# Autodesk Inventor assembly: Roller Assembly 1764
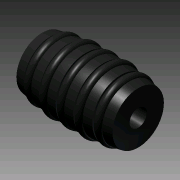
[picture p0: Inventor's stored thumbnail of the model, 180x180]
Saved by Autodesk Inventor 2011 (Build 150239000, 239)
## iProperties
Created: 2007-11-29
Part Number: Roller Assembly 1764
Document SubType Name: Assembly
Designer: lwoods
Author: lwoods
## Documents named in this file (4)
- R:\CAD Archives\Wheels\Omniwheel 1764\Roller Assembly 1764.iam
- R:\CAD Archives\Wheels\Omniwheel 1764\RollerRidges 1764.ipt
- R:\CAD Archives\Wheels\Omniwheel 1764\O Ring 1 R.609 1764.ipt
- R:\CAD Archives\Wheels\Omniwheel 1764\O Ring 2 R.671 1764.ipt
## Components (6 placed, 3 different names)
1. RollerRidges 1764:1 — Mate:2, Mate:7, Mate:11, Mate:16, Mate:19, Mate:25
2. O Ring 1 R.609 1764:1 — Mate:4, Angle:1, Mate:6
3. O Ring 1 R.609 1764:2 — Mate:8, Angle:2, Mate:9
4. O Ring 2 R.671 1764:1 — Mate:13, Angle:3, Mate:14
5. O Ring 2 R.671 1764:2 — Mate:12, Angle:4, Mate:17
6. O Ring 2 R.671 1764:3 — Mate:20, Angle:6, Mate:23
## Relationships (27: Mate 22, Angle 5)
- Mate:2: RollerRidges 1764:1
- Mate:3
- Mate:4: O Ring 1 R.609 1764:1
- Mate:5
- Angle:1 (0 deg): O Ring 1 R.609 1764:1
- Mate:6: O Ring 1 R.609 1764:1
- Mate:7 (-4.8666 mm): RollerRidges 1764:1
- Mate:8: O Ring 1 R.609 1764:2
- Angle:2 (0 deg): O Ring 1 R.609 1764:2
- Mate:9: O Ring 1 R.609 1764:2
- Mate:10
- Mate:11 (-4.8666 mm): RollerRidges 1764:1
- Mate:12: O Ring 2 R.671 1764:2
- Mate:13: O Ring 2 R.671 1764:1
- Angle:3 (0 deg): O Ring 2 R.671 1764:1
- Mate:14: O Ring 2 R.671 1764:1
- Mate:15
- Mate:16 (1.5875 mm): RollerRidges 1764:1
- Angle:4 (0 deg): O Ring 2 R.671 1764:2
- Mate:17: O Ring 2 R.671 1764:2
- Mate:18
- Mate:19 (1.5875 mm): RollerRidges 1764:1
- Mate:20: O Ring 2 R.671 1764:3
- Angle:6 (0 deg): O Ring 2 R.671 1764:3
- Mate:23: O Ring 2 R.671 1764:3
- Mate:24
- Mate:25 (1.5875 mm): RollerRidges 1764:1
